# Autodesk Inventor assembly: Y-axis Frame Return assy
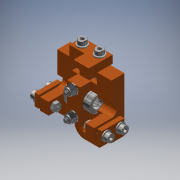
[picture p0: Inventor's stored thumbnail of the model, 180x180]
Saved by Autodesk Inventor 2018 (Build 220112000, 112)
## iProperties
Created: 2017-10-03
Part Number: Y-axis Frame Return assy
Document SubType Name: Assembly
Designer: Gabriel Smolnycki
Author: Gabriel Smolnycki
## Documents named in this file (13)
- H:\dev\planb\mechanics\V1INV\Subassemblies\Y-axis Frame Return assy.iam
- H:\dev\planb\mechanics\V1INV\Y-axis\Y-axis Frame Block.ipt
- H:\dev\planb\mechanics\V1INV\Y-axis\Y-axis Belt Return.ipt
- H:\dev\planb\mechanics\V1INV\Y-axis\Y-axis Linear Bearing Clamp.ipt
- H:\dev\planb\mechanics\V1INV\Hardware\8x25 Linear Bearing (63255K45).ipt
- H:\dev\planb\mechanics\V1INV\Hardware\M4 SS Washer.ipt
- H:\dev\planb\mechanics\V1INV\Hardware\M4 SS Locknut.ipt
- H:\dev\planb\mechanics\V1INV\Hardware\M4x35 SS SHCS.ipt
- H:\dev\planb\mechanics\V1INV\Hardware\M4 SS Nut.ipt
- H:\dev\planb\mechanics\V1INV\Hardware\M4x20 SS SHCS.ipt
- H:\dev\planb\mechanics\V1INV\Y-axis\Y-axis Belt Clamp.ipt
- H:\dev\planb\mechanics\V1INV\Hardware\M4x16 SS SHCS.ipt
- H:\dev\planb\mechanics\V1INV\Hardware\4x13 SS Ball Bearing (7804K103).ipt
## Components (41 placed, 12 different names)
1. Y-axis Frame Block:1 — Insert:1, Insert:2, Insert:3, Insert:4, Insert:5, Insert:14, Insert:15, Mate:1, Mate:2, Mate:3, Mate:4, Insert:16, Insert:17, Insert:20, Insert:21, Insert:22, Insert:23, Mate:5, Mate:6, Mate:7, Mate:8, Insert:28, Insert:29, Insert:34, Insert:35, Insert:36, Mate:9, Insert:37
2. Y-axis Belt Return:1 — Insert:4, Insert:5, Insert:6, Insert:7, Insert:38, Insert:39, Insert:40, Insert:41, Insert:43
3. Y-axis Linear Bearing Clamp:1 — Insert:2, Insert:3, Insert:8, Insert:9
4. 8x25 Linear Bearing (63255K45):1 — Insert:1
5. M4 SS Washer:1 — Insert:6
6. M4 SS Washer:2 — Insert:7
7. M4 SS Washer:3 — Insert:8, Insert:10
8. M4 SS Washer:4 — Insert:9, Insert:11
9. M4 SS Locknut:1 — Insert:10
10. M4 SS Locknut:2 — Insert:11
11. M4x35 SS SHCS:1
12. M4x35 SS SHCS:2
13. M4 SS Nut:1 — Mate:3, Mate:4, Insert:17
14. M4 SS Nut:2 — Mate:1, Mate:2, Insert:16
15. M4 SS Washer:5 — Insert:14, Insert:18
16. M4 SS Washer:6 — Insert:15, Insert:19
17. M4x20 SS SHCS:1 — Insert:18
18. M4x20 SS SHCS:2 — Insert:19
19. M4 SS Nut:3 — Insert:20, Mate:7
20. M4 SS Nut:4 — Insert:21, Mate:8
21. M4 SS Nut:5 — Insert:22, Mate:5
22. M4 SS Nut:6 — Insert:23, Mate:6
23. Y-axis Belt Clamp:1 — Insert:24, Insert:25, Insert:28, Insert:29
24. M4 SS Washer:7 — Insert:24, Insert:26
25. M4 SS Washer:8 — Insert:25, Insert:27
26. M4x20 SS SHCS:3 — Insert:26
27. M4x20 SS SHCS:4 — Insert:27
28. Y-axis Belt Clamp:2 — Insert:34, Insert:35
29. M4 SS Washer:9
30. M4 SS Washer:10
31. M4x20 SS SHCS:5
32. M4x20 SS SHCS:6
33. M4x16 SS SHCS:1 — Insert:37
34. M4 SS Nut:7 — Insert:36, Mate:9
35. M4 SS Washer:11 — Insert:38, Insert:44
36. M4 SS Washer:12 — Insert:39
37. M4 SS Washer:13 — Insert:40
38. M4 SS Washer:14 — Insert:41, Insert:42
39. M4x20 SS SHCS:7 — Insert:44
40. 4x13 SS Ball Bearing (7804K103):1 — Insert:43
41. M4 SS Locknut:3 — Insert:42
## Relationships (53: Insert 44, Mate 9)
- Insert:1 (0.25 mm): Y-axis Frame Block:1 ↔ 8x25 Linear Bearing (63255K45):1
- Insert:2: Y-axis Frame Block:1 ↔ Y-axis Linear Bearing Clamp:1
- Insert:3: Y-axis Frame Block:1 ↔ Y-axis Linear Bearing Clamp:1
- Insert:4: Y-axis Frame Block:1 ↔ Y-axis Belt Return:1
- Insert:5: Y-axis Frame Block:1 ↔ Y-axis Belt Return:1
- Insert:6: Y-axis Belt Return:1 ↔ M4 SS Washer:1
- Insert:7: Y-axis Belt Return:1 ↔ M4 SS Washer:2
- Insert:8: Y-axis Linear Bearing Clamp:1 ↔ M4 SS Washer:3
- Insert:9: Y-axis Linear Bearing Clamp:1 ↔ M4 SS Washer:4
- Insert:10: M4 SS Washer:3 ↔ M4 SS Locknut:1
- Insert:11: M4 SS Washer:4 ↔ M4 SS Locknut:2
- [Insert]: M4 SS Washer:1 ↔ M4x35 SS SHCS:1
- [Insert]: M4 SS Washer:2 ↔ M4x35 SS SHCS:2
- Insert:14: Y-axis Frame Block:1 ↔ M4 SS Washer:5
- Insert:15: Y-axis Frame Block:1 ↔ M4 SS Washer:6
- Mate:1: Y-axis Frame Block:1 ↔ M4 SS Nut:2
- Mate:2: Y-axis Frame Block:1 ↔ M4 SS Nut:2
- Mate:3: Y-axis Frame Block:1 ↔ M4 SS Nut:1
- Mate:4: Y-axis Frame Block:1 ↔ M4 SS Nut:1
- Insert:16: Y-axis Frame Block:1 ↔ M4 SS Nut:2
- Insert:17: Y-axis Frame Block:1 ↔ M4 SS Nut:1
- Insert:18: M4 SS Washer:5 ↔ M4x20 SS SHCS:1
- Insert:19: M4 SS Washer:6 ↔ M4x20 SS SHCS:2
- Insert:20: Y-axis Frame Block:1 ↔ M4 SS Nut:3
- Insert:21: Y-axis Frame Block:1 ↔ M4 SS Nut:4
- Insert:22: Y-axis Frame Block:1 ↔ M4 SS Nut:5
- Insert:23: Y-axis Frame Block:1 ↔ M4 SS Nut:6
- Mate:5: Y-axis Frame Block:1 ↔ M4 SS Nut:5
- Mate:6: Y-axis Frame Block:1 ↔ M4 SS Nut:6
- Mate:7: Y-axis Frame Block:1 ↔ M4 SS Nut:3
- Mate:8: Y-axis Frame Block:1 ↔ M4 SS Nut:4
- Insert:24: Y-axis Belt Clamp:1 ↔ M4 SS Washer:7
- Insert:25: Y-axis Belt Clamp:1 ↔ M4 SS Washer:8
- Insert:26: M4 SS Washer:7 ↔ M4x20 SS SHCS:3
- Insert:27: M4 SS Washer:8 ↔ M4x20 SS SHCS:4
- Insert:28 (2 mm): Y-axis Frame Block:1 ↔ Y-axis Belt Clamp:1
- Insert:29: Y-axis Frame Block:1 ↔ Y-axis Belt Clamp:1
- [Insert]: Y-axis Belt Clamp:2 ↔ M4 SS Washer:9
- [Insert]: Y-axis Belt Clamp:2 ↔ M4 SS Washer:10
- [Insert]: M4 SS Washer:9 ↔ M4x20 SS SHCS:5
- [Insert]: M4 SS Washer:10 ↔ M4x20 SS SHCS:6
- Insert:34 (2 mm): Y-axis Frame Block:1 ↔ Y-axis Belt Clamp:2
- Insert:35: Y-axis Frame Block:1 ↔ Y-axis Belt Clamp:2
- Insert:36: Y-axis Frame Block:1 ↔ M4 SS Nut:7
- Mate:9: Y-axis Frame Block:1 ↔ M4 SS Nut:7
- Insert:37: Y-axis Frame Block:1 ↔ M4x16 SS SHCS:1
- Insert:38: Y-axis Belt Return:1 ↔ M4 SS Washer:11
- Insert:39: Y-axis Belt Return:1 ↔ M4 SS Washer:12
- Insert:40: Y-axis Belt Return:1 ↔ M4 SS Washer:13
- Insert:41: Y-axis Belt Return:1 ↔ M4 SS Washer:14
- Insert:42: M4 SS Washer:14 ↔ M4 SS Locknut:3
- Insert:43 (0.5 mm): Y-axis Belt Return:1 ↔ 4x13 SS Ball Bearing (7804K103):1
- Insert:44: M4 SS Washer:11 ↔ M4x20 SS SHCS:7
## Named parameters: d39_d31 = 0 mm, d40_d32 = 0 mm, d41_d33 = 0 mm, d42_d34 = 0 mm
